# Autodesk Inventor assembly: Engine Assembly
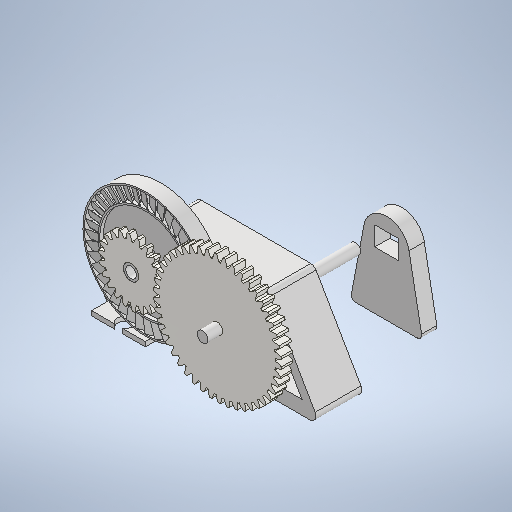
[picture p0: Inventor's stored thumbnail of the model, 512x512]
Saved by Autodesk Inventor 2026.1 (Build 301233020, 233B)
## iProperties
Created: 2025-11-03
Part Number: Engine Assembly
Document SubType Name: Assembly
Designer: yo
Author: yo
## Documents named in this file (6)
- C:\Users\yo\Documents\Andes\9no Semestre\Proyecto Intermedio\Proyecto\Huron-Hudson\Pelton Engine\V10\Engine Assembly.iam
- C:\Users\yo\Documents\Andes\9no Semestre\Proyecto Intermedio\Proyecto\Huron-Hudson\Pelton Engine\V10\EngineMount - Big hole.ipt
- C:\Users\yo\Documents\Andes\9no Semestre\Proyecto Intermedio\Proyecto\Huron-Hudson\Pelton Engine\V10\Impulse Turbine 2.ipt
- C:\Users\yo\Documents\Andes\9no Semestre\Proyecto Intermedio\Proyecto\Huron-Hudson\Pelton Engine\V10\Shaft.ipt
- C:\Users\yo\Documents\Andes\9no Semestre\Proyecto Intermedio\Proyecto\Huron-Hudson\Pelton Engine\V10\Engine Assembly\Design Accelerator\Spur Gears1.iam
- C:\Users\yo\Documents\Andes\9no Semestre\Proyecto Intermedio\Proyecto\Huron-Hudson\Pelton Engine\V10\Sensor Stand.ipt
## Components (5 placed, 5 different names)
1. EngineMount - Big hole:1 — Flush:1, Flush:2, Flush:3, Mate:1, Tangent:1, Mate:2
2. Impulse Turbine 2:1 — Mate:1, Tangent:1, Mate:3, Mate:4, Mate:6
3. Shaft:1 — Mate:2, Flush:4, Mate:5
4. Spur Gears:1 [sub-assembly] — Mate:3, Mate:4, Mate:5, Mate:6
5. Sensor Stand:1 — Flush:5
## Relationships (12: Mate 6, Flush 5, Tangent 1)
- Flush:1: EngineMount - Big hole:1
- Flush:2: EngineMount - Big hole:1
- Flush:3: EngineMount - Big hole:1
- Mate:1: EngineMount - Big hole:1 ↔ Impulse Turbine 2:1
- Tangent:1: EngineMount - Big hole:1 ↔ Impulse Turbine 2:1
- Mate:2: EngineMount - Big hole:1 ↔ Shaft:1
- Flush:4: Shaft:1
- Mate:3: Impulse Turbine 2:1 ↔ Spur Gears:1
- Mate:4: Impulse Turbine 2:1 ↔ Spur Gears:1
- Mate:5: Shaft:1 ↔ Spur Gears:1
- Mate:6: Impulse Turbine 2:1 ↔ Spur Gears:1
- Flush:5: Sensor Stand:1
